# Autodesk Inventor assembly: Collection assembly
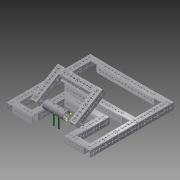
[picture p0: Inventor's stored thumbnail of the model, 180x180]
Saved by Autodesk Inventor 2015 (Build 190159000, 159)
## iProperties
Created: 2014-11-17
Part Number: Collection assembly
Document SubType Name: Assembly
Designer: lethcoec
Author: lethcoec
## Documents named in this file (3)
- \\st-svr\studenthdrives$\18\LethcoeC\FTC Cascade effect\Collection assembly.iam
- \\st-svr\studenthdrives$\18\LethcoeC\FTC Cascade effect\FTC ROBOT DRIVE TRAIN.iam
- \\st-svr\studenthdrives$\18\LethcoeC\FTC Cascade effect\Imported Components\Channel160mm\Channel160mm.ipt
## Components (4 placed, 2 different names)
1. FTC ROBOT DRIVE TRAIN:1 [sub-assembly] — Mate:1, Mate:2
2. Channel160mm:1 — Mate:2, Flush:1, Flush:2
3. Channel160mm:2 — Mate:1, Mate:3
4. Channel160mm:3 — Mate:3, Flush:1, Flush:2
## Relationships (5: Mate 3, Flush 2)
- Mate:1: FTC ROBOT DRIVE TRAIN:1 ↔ Channel160mm:2
- Mate:2: FTC ROBOT DRIVE TRAIN:1 ↔ Channel160mm:1
- Mate:3: Channel160mm:2 ↔ Channel160mm:3
- Flush:1: Channel160mm:1 ↔ Channel160mm:3
- Flush:2: Channel160mm:1 ↔ Channel160mm:3
